# Autodesk Inventor assembly: side of drivetrain
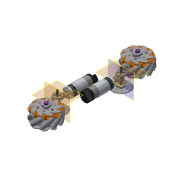
[picture p0: Inventor's stored thumbnail of the model, 180x180]
Saved by Autodesk Inventor 2019 (Build 230136000, 136)
## iProperties
Created: 2019-10-04
Part Number: side of drivetrain
Document SubType Name: Assembly
Designer: ball
Author: ball
## Documents named in this file (1)
- C:\FTC\FTC8863CAD\2019 Robot\Mecanum Drive Train\side of drivetrain.iam
## Components (2 placed, 2 different names)
1. wheel with drive motor top:1 [sub-assembly] — Mate:1, Flush:4, Mate:2
2. wheel with drive motor floor:1 [sub-assembly] — Mate:1, Flush:4, Mate:2
## Relationships (3: Mate 2, Flush 1)
- Mate:1 (349.25 mm): wheel with drive motor top:1 ↔ wheel with drive motor floor:1
- Flush:4: wheel with drive motor top:1 ↔ wheel with drive motor floor:1
- Mate:2: wheel with drive motor top:1 ↔ wheel with drive motor floor:1
